# Autodesk Inventor assembly: corner tab
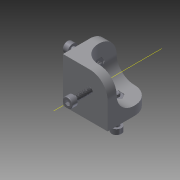
[picture p0: Inventor's stored thumbnail of the model, 180x180]
Saved by Autodesk Inventor 2014 (Build 180170000, 170)
## iProperties
Created: 2013-10-14
Part Number: corner tab
Document SubType Name: Assembly
Designer: employee
Author: employee
## Documents named in this file (4)
- \\GRISTLE\speco\GitHub\ConceptFORGE\Wally\corner tab.iam
- \\GRISTLE\speco\GitHub\ConceptFORGE\Wally\corner tab.ipt
- \\GRISTLE\speco\GitHub\ConceptFORGE\Wally\m3 nut.ipt
- \\GRISTLE\speco\GitHub\ConceptFORGE\Wally\M3x16.ipt
## Components (7 placed, 3 different names)
1. corner tab:1 — Insert:1, Insert:2, Insert:3, Angle:1, Angle:2, Angle:3, Insert:4, Insert:5, Insert:6
2. Hex Nut Metric M3 x 0.5:1 — Insert:1, Angle:3
3. Hex Nut Metric M3 x 0.5:2 — Insert:3, Angle:1
4. Hex Nut Metric M3 x 0.5:3 — Insert:2, Angle:2
5. Forged Socket Head Cap Screw - Metric M3x0.5 x 16:1 — Insert:4
6. Forged Socket Head Cap Screw - Metric M3x0.5 x 16:2 — Insert:5
7. Forged Socket Head Cap Screw - Metric M3x0.5 x 16:3 — Insert:6
## Relationships (9: Insert 6, Angle 3)
- Insert:1: corner tab:1 ↔ Hex Nut Metric M3 x 0.5:1
- Insert:2: corner tab:1 ↔ Hex Nut Metric M3 x 0.5:3
- Insert:3: corner tab:1 ↔ Hex Nut Metric M3 x 0.5:2
- Angle:1 (0 deg): corner tab:1 ↔ Hex Nut Metric M3 x 0.5:2
- Angle:2 (0 deg): corner tab:1 ↔ Hex Nut Metric M3 x 0.5:3
- Angle:3 (0 deg): corner tab:1 ↔ Hex Nut Metric M3 x 0.5:1
- Insert:4 (9.5 mm): corner tab:1 ↔ Forged Socket Head Cap Screw - Metric M3x0.5 x 16:1
- Insert:5 (9.5 mm): corner tab:1 ↔ Forged Socket Head Cap Screw - Metric M3x0.5 x 16:2
- Insert:6 (9.5 mm): corner tab:1 ↔ Forged Socket Head Cap Screw - Metric M3x0.5 x 16:3
